# Autodesk Inventor assembly: M2-タミヤダンパー1
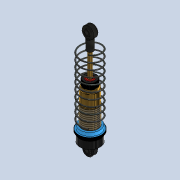
[picture p0: Inventor's stored thumbnail of the model, 180x180]
Saved by Autodesk Inventor 2020 (Build 240168000, 168)
## iProperties
Part Number: M2-タミヤダンパー1
Material: 一般
Document SubType Name: Assembly
Designer: AA19065
Mass: 70.809 g
Surface Area: 76.0005 cm^2
Volume: 5.68479 cm^3
Density: 12.4559 g/cm^3
Author: 雪村
## Documents named in this file (10)
- C:\Users\happy\OneDrive\ドキュメント\賢一ファイル\SRDC\試作10-2\アセンブリ\M2-タミヤダンパー1.iam
- C:\Users\happy\OneDrive\ドキュメント\賢一ファイル\SRDC\試作10-2\ダンパ\M2-タミヤダンパー1.ipt
- C:\Users\happy\OneDrive\ドキュメント\賢一ファイル\SRDC\試作10-2\ダンパ\M2-タミヤダンパー2.ipt
- C:\Users\happy\OneDrive\ドキュメント\賢一ファイル\SRDC\試作10-2\ダンパ\M2-タミヤダンパー3.ipt
- C:\Users\happy\OneDrive\ドキュメント\賢一ファイル\SRDC\試作10-2\ダンパ\M2-タミヤダンパー4.ipt
- C:\Users\happy\OneDrive\ドキュメント\賢一ファイル\SRDC\試作10-2\ダンパ\M2-タミヤダンパー6.ipt
- C:\Users\happy\OneDrive\ドキュメント\賢一ファイル\SRDC\試作10-2\ダンパ\M2-タミヤダンパー5.ipt
- C:\Users\happy\OneDrive\ドキュメント\賢一ファイル\SRDC\試作10-2\ダンパ\M2-タミヤダンパー7.ipt
- C:\Users\happy\OneDrive\ドキュメント\賢一ファイル\SRDC\試作10-2\ダンパ\M2-タミヤダンパー8.ipt
- C:\Users\happy\OneDrive\ドキュメント\賢一ファイル\SRDC\試作10-2\ダンパ\M2-タミヤダンパー9.ipt
## Components (10 placed, 9 different names)
1. M2-タミヤダンパー1:1 — 挿入:1, フラッシュ:1, フラッシュ:3, ボール:2
2. M2-タミヤダンパー2:1 — 挿入:1, 挿入:2, メイト:1, 円柱状:2
3. M2-タミヤダンパー3:1 — 挿入:2, 挿入:3
4. M2-タミヤダンパー4:1 — メイト:1, 円柱状:2
5. M2-タミヤダンパー6:1 — 挿入:3, メイト:2
6. M2-タミヤダンパー5:1 — メイト:2, 挿入:4, メイト:3
7. M2-タミヤダンパー7:1 — フラッシュ:1, 挿入:4
8. M2-タミヤダンパー8:1 — フラッシュ:3, フラッシュ:2, ボール:2
9. M2-タミヤダンパー8:2 — フラッシュ:2
10. M2-タミヤダンパー9:1 — メイト:3
## Relationships (12: Insert 4, Mate 3, Flush 3, CylindricalJoint 1, BallJoint 1)
- 挿入:1 [Insert]: M2-タミヤダンパー1:1 ↔ M2-タミヤダンパー2:1
- 挿入:2 [Insert]: M2-タミヤダンパー2:1 ↔ M2-タミヤダンパー3:1
- メイト:1 [Mate]: M2-タミヤダンパー2:1 ↔ M2-タミヤダンパー4:1
- 挿入:3 [Insert]: M2-タミヤダンパー3:1 ↔ M2-タミヤダンパー6:1
- メイト:2 [Mate]: M2-タミヤダンパー6:1 ↔ M2-タミヤダンパー5:1
- フラッシュ:1 [Flush]: M2-タミヤダンパー1:1 ↔ M2-タミヤダンパー7:1
- 挿入:4 [Insert] (-3 mm): M2-タミヤダンパー5:1 ↔ M2-タミヤダンパー7:1
- フラッシュ:3 [Flush]: M2-タミヤダンパー1:1 ↔ M2-タミヤダンパー8:1
- フラッシュ:2 [Flush]: M2-タミヤダンパー8:1 ↔ M2-タミヤダンパー8:2
- メイト:3 [Mate]: M2-タミヤダンパー5:1 ↔ M2-タミヤダンパー9:1
- 円柱状:2 [CylindricalJoint]: M2-タミヤダンパー2:1 ↔ M2-タミヤダンパー4:1
- ボール:2 [BallJoint]: M2-タミヤダンパー1:1 ↔ M2-タミヤダンパー8:1
